# Autodesk Inventor assembly: Wiping machine
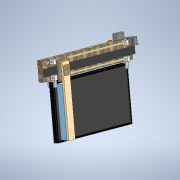
[picture p0: Inventor's stored thumbnail of the model, 180x180]
Saved by Autodesk Inventor 2020 (Build 240168000, 168)
## iProperties
Created: 2021-07-09
Part Number: Wiping machine
Document SubType Name: Assembly
Designer: pc
Author: pc
## Documents named in this file (14)
- C:\Users\pc\Documents\Wiping machine.iam
- C:\Users\pc\Documents\support1.ipt
- C:\Users\pc\Documents\nut.ipt
- C:\Users\pc\Documents\rod1.ipt
- C:\Users\pc\Documents\nema 23 stepper.ipt
- C:\Users\pc\Documents\belt axle.ipt
- C:\Users\pc\Documents\belt.ipt
- C:\Users\pc\Documents\attach.ipt
- C:\Users\pc\Documents\Battery1.ipt
- C:\Users\pc\Documents\Button.ipt
- C:\Users\pc\Documents\slider.ipt
- C:\Users\pc\Documents\blade.ipt
- C:\Users\pc\Documents\tv1.ipt
- C:\Users\pc\Documents\Cloth.ipt
## Components (18 placed, 13 different names)
1. nut:1 — Mate:1, Mate:3, Mate:11, Flush:4, Flush:8
2. nut:2 — Mate:2, Mate:4, Mate:12, Flush:3, Flush:7
3. nut:3 — Mate:6, Mate:7, Mate:10, Flush:1, Flush:7, Mate:34
4. nut:4 — Mate:5, Mate:8, Mate:9, Flush:2, Flush:8
5. rod1:1 — Mate:1, Mate:2, Mate:3, Mate:4, Mate:41
6. rod1:2 — Mate:5, Mate:6, Mate:7, Mate:8, Mate:40
7. nema 23 stepper:1 — Mate:13, Mate:30
8. support1:1 — Mate:9, Mate:10, Flush:1, Flush:2, Mate:11, Mate:12, Flush:3, Flush:4, Mate:13, Mate:14, Flush:6, Mate:24, Flush:16, Mate:31, Flush:21, Mate:32, Mate:42
9. belt axle:1 — Mate:14, Flush:6, Mate:15
10. belt:1 — Mate:15, Mate:30
11. attach:2 — Mate:24, Flush:16, Mate:39, Flush:23
12. Battery1:1 — Mate:31, Flush:21
13. Button:2 — Mate:32
14. slider:1 — Mate:34, Mate:35, Mate:36, Mate:37, Flush:22, Mate:40, Mate:41
15. blade:1 — Mate:35, Mate:36, Mate:37, Flush:22, Mate:43, Flush:25, Flush:26
16. tv1:1 — Mate:39, Flush:23, Flush:24
17. attach:3 — Mate:42, Flush:24
18. Cloth:1 — Mate:43, Flush:25, Flush:26
## Relationships (42: Mate 28, Flush 14)
- Mate:1: nut:1 ↔ rod1:1
- Mate:2: nut:2 ↔ rod1:1
- Mate:3: nut:1 ↔ rod1:1
- Mate:4: nut:2 ↔ rod1:1
- Mate:5: nut:4 ↔ rod1:2
- Mate:6: nut:3 ↔ rod1:2
- Mate:7: nut:3 ↔ rod1:2
- Mate:8: nut:4 ↔ rod1:2
- Mate:9: nut:4 ↔ support1:1
- Mate:10: nut:3 ↔ support1:1
- Flush:1: nut:3 ↔ support1:1
- Flush:2: nut:4 ↔ support1:1
- Mate:11: nut:1 ↔ support1:1
- Mate:12: nut:2 ↔ support1:1
- Flush:3: nut:2 ↔ support1:1
- Flush:4: nut:1 ↔ support1:1
- Mate:13: nema 23 stepper:1 ↔ support1:1
- Mate:14: support1:1 ↔ belt axle:1
- Flush:6: support1:1 ↔ belt axle:1
- Flush:7: nut:2 ↔ nut:3
- Flush:8: nut:1 ↔ nut:4
- Mate:15: belt axle:1 ↔ belt:1
- Mate:24: support1:1 ↔ attach:2
- Flush:16: support1:1 ↔ attach:2
- Mate:30: nema 23 stepper:1 ↔ belt:1
- Mate:31: support1:1 ↔ Battery1:1
- Flush:21: support1:1 ↔ Battery1:1
- Mate:32: support1:1 ↔ Button:2
- Mate:34: nut:3 ↔ slider:1
- Mate:35: slider:1 ↔ blade:1
- Mate:36: slider:1 ↔ blade:1
- Mate:37: slider:1 ↔ blade:1
- Flush:22: slider:1 ↔ blade:1
- Mate:39: attach:2 ↔ tv1:1
- Mate:40 (25.4 mm): rod1:2 ↔ slider:1
- Mate:41 (25.4 mm): rod1:1 ↔ slider:1
- Mate:42: support1:1 ↔ attach:3
- Mate:43: blade:1 ↔ Cloth:1
- Flush:23: attach:2 ↔ tv1:1
- Flush:24: tv1:1 ↔ attach:3
- Flush:25: blade:1 ↔ Cloth:1
- Flush:26: blade:1 ↔ Cloth:1
